# Autodesk Inventor assembly: bed
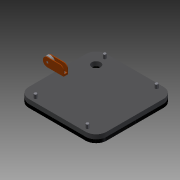
[picture p0: Inventor's stored thumbnail of the model, 180x180]
Saved by Autodesk Inventor 2013 (Build 170138000, 138)
## iProperties
Created: 2013-10-14
Part Number: bed
Document SubType Name: Assembly
Designer: employee
Author: employee
## Documents named in this file (12)
- C:\Users\employee\Desktop\new wally\bed.iam
- C:\Users\employee\Desktop\new wally\bed.ipt
- C:\Users\employee\Desktop\new wally\hot bed.ipt
- C:\Users\employee\Desktop\new wally\M3x16.ipt
- C:\Users\employee\Desktop\new wally\z pulley holder.ipt
- C:\Users\employee\Desktop\new wally\m3 nut.ipt
- C:\Users\employee\Desktop\new wally\M3x10.ipt
- C:\Users\employee\Desktop\new wally\608.ipt
- C:\Users\employee\Desktop\new wally\basalt.ipt
- C:\Users\employee\Desktop\new wally\M8x35.ipt
- C:\Users\employee\Desktop\new wally\plastic washer.ipt
- C:\Users\employee\Desktop\new wally\z idler.ipt
## Components (20 placed, 11 different names)
1. bed:1 — Insert:1, Insert:2, Insert:3, Insert:6, Insert:7, Insert:11, Insert:12
2. hot bed:1 — Insert:3
3. Forged Socket Head Cap Screw - Metric M3x0.5 x 16:1 — Insert:1
4. Forged Socket Head Cap Screw - Metric M3x0.5 x 16:2 — Insert:2
5. z pulley holder:1 — Insert:4, Insert:5, Angle:1, Angle:2, Insert:6, Insert:7, Insert:8, Insert:9, Angle:3, Insert:10
6. Hex Nut Metric M3 x 0.5:1 — Insert:4, Angle:1
7. Hex Nut Metric M3 x 0.5:2 — Insert:5, Angle:2
8. M3x10:1 — Insert:8
9. Hex Nut Metric M3 x 0.5:3 — Insert:9, Angle:3
10. 608:1 — Insert:10, Insert:21
11. basalt:1 — Insert:11, Insert:12, Insert:13, Insert:14, Insert:15, Insert:16
12. Hex Bolt - Metric M8 x 1.25 x 35:1 — Insert:20
13. Hex Bolt - Metric M8 x 1.25 x 35:2 — Insert:19
14. Hex Bolt - Metric M8 x 1.25 x 35:3 — Insert:18
15. Hex Bolt - Metric M8 x 1.25 x 35:4 — Insert:17
16. plastic washer:1 — Insert:13, Insert:19
17. plastic washer:2 — Insert:14, Insert:18
18. plastic washer:3 — Insert:15, Insert:20
19. plastic washer:4 — Insert:16, Insert:17
20. z idler:1 — Insert:21
## Relationships (24: Insert 21, Angle 3)
- Insert:1: bed:1 ↔ Forged Socket Head Cap Screw - Metric M3x0.5 x 16:1
- Insert:2: bed:1 ↔ Forged Socket Head Cap Screw - Metric M3x0.5 x 16:2
- Insert:3: bed:1 ↔ hot bed:1
- Insert:4: z pulley holder:1 ↔ Hex Nut Metric M3 x 0.5:1
- Insert:5: z pulley holder:1 ↔ Hex Nut Metric M3 x 0.5:2
- Angle:1 (0 deg): z pulley holder:1 ↔ Hex Nut Metric M3 x 0.5:1
- Angle:2 (0 deg): z pulley holder:1 ↔ Hex Nut Metric M3 x 0.5:2
- Insert:6: bed:1 ↔ z pulley holder:1
- Insert:7: bed:1 ↔ z pulley holder:1
- Insert:8: z pulley holder:1 ↔ M3x10:1
- Insert:9: z pulley holder:1 ↔ Hex Nut Metric M3 x 0.5:3
- Angle:3 (0 deg): z pulley holder:1 ↔ Hex Nut Metric M3 x 0.5:3
- Insert:10: z pulley holder:1 ↔ 608:1
- Insert:11: bed:1 ↔ basalt:1
- Insert:12: bed:1 ↔ basalt:1
- Insert:13: basalt:1 ↔ plastic washer:1
- Insert:14: basalt:1 ↔ plastic washer:2
- Insert:15: basalt:1 ↔ plastic washer:3
- Insert:16: basalt:1 ↔ plastic washer:4
- Insert:17: Hex Bolt - Metric M8 x 1.25 x 35:4 ↔ plastic washer:4
- Insert:18: Hex Bolt - Metric M8 x 1.25 x 35:3 ↔ plastic washer:2
- Insert:19: Hex Bolt - Metric M8 x 1.25 x 35:2 ↔ plastic washer:1
- Insert:20: Hex Bolt - Metric M8 x 1.25 x 35:1 ↔ plastic washer:3
- Insert:21: 608:1 ↔ z idler:1
